# Autodesk Inventor assembly: Katamaran
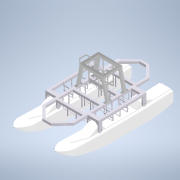
[picture p0: Inventor's stored thumbnail of the model, 180x180]
Saved by Autodesk Inventor 2020 (Build 240168000, 168)
## iProperties
Created: 2020-05-27
Part Number: Katamaran
Document SubType Name: Assembly
Designer: Chris
Author: Chris
## Documents named in this file (4)
- C:\Users\Chris\Desktop\Masterarbeit\CAD\Katamaran.iam
- C:\Users\Chris\Desktop\Masterarbeit\CAD\Rahmen_neu.ipt
- C:\Users\Chris\Desktop\Masterarbeit\CAD\Kufe.ipt
- C:\Users\Chris\Desktop\Masterarbeit\CAD\zweite_Ebene.ipt
## Components (4 placed, 3 different names)
1. Rahmen:1 — Passend:1, Passend:2, Passend:3, Passend:4, Passend:5, Fluchtend:1, Fluchtend:2
2. Kufe:1 — Passend:4
3. Kufe:2 — Passend:1, Passend:2, Passend:3
4. zweite_Ebene:1 — Passend:5, Fluchtend:1, Fluchtend:2
## Relationships (7: Mate 5, Flush 2)
- Passend:1 [Mate]: Rahmen:1 ↔ Kufe:2
- Passend:2 [Mate]: Rahmen:1 ↔ Kufe:2
- Passend:3 [Mate]: Rahmen:1 ↔ Kufe:2
- Passend:4 [Mate]: Rahmen:1 ↔ Kufe:1
- Passend:5 [Mate]: Rahmen:1 ↔ zweite_Ebene:1
- Fluchtend:1 [Flush]: Rahmen:1 ↔ zweite_Ebene:1
- Fluchtend:2 [Flush] (700 mm): Rahmen:1 ↔ zweite_Ebene:1
